# Autodesk Inventor assembly: main_sim
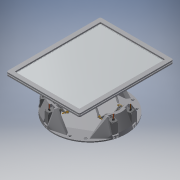
[picture p0: Inventor's stored thumbnail of the model, 180x180]
Saved by Autodesk Inventor 2017 (Build 210142000, 142)
## iProperties
Part Number: main_sim
Material: Ogólny
Document SubType Name: Assembly
Designer: Peter
Author: Peter
## Documents named in this file (5)
- F:\Workspace\Inventor\Ti\CAD\model\Sim assembly\main_sim.iam
- F:\Workspace\Inventor\Ti\CAD\model\Sim assembly\section_lever_sim.ipt
- F:\Workspace\Inventor\Ti\CAD\model\Sim assembly\section_middle_sim.ipt
- F:\Workspace\Inventor\Ti\CAD\model\Sim assembly\section_rod_sim.ipt
- F:\Workspace\Inventor\Ti\CAD\model\Sim assembly\section_upper_sim.ipt
## Components (14 placed, 4 different names)
1. section_middle_sim:1 — Równoległy:2, Równoległy:3, Równoległy:1, Zestawiający:7, Zestawiający:8, Zestawiający:11, Zestawiający:12, Zestawiający:14, Zestawiający:15, Zestawiający:16, Zestawiający:17, Zestawiający:18, Zestawiający:19, Zestawiający:20, Zestawiający:21, Kąt:1, Kąt:2, Kąt:3, Kąt:4, Kąt:5, Kąt:6
2. section_lever_sim:1 — Zestawiający:20, Zestawiający:21, Kąt:1, Zestawiający:22
3. section_lever_sim:2 — Zestawiający:7, Zestawiający:8, Kąt:2, Zestawiający:23
4. section_lever_sim:3 — Zestawiający:11, Zestawiający:12, Kąt:3, Zestawiający:24
5. section_lever_sim:4 — Zestawiający:14, Zestawiający:15, Kąt:4, Zestawiający:25
6. section_lever_sim:5 — Zestawiający:16, Zestawiający:17, Kąt:5, Zestawiający:26
7. section_lever_sim:6 — Zestawiający:18, Zestawiający:19, Kąt:6, Zestawiający:27
8. section_rod_sim:1 — Zestawiający:22, Zestawiający:28
9. section_rod_sim:2 — Zestawiający:23, Zestawiający:29
10. section_rod_sim:3 — Zestawiający:24, Zestawiający:30
11. section_rod_sim:4 — Zestawiający:25, Zestawiający:31
12. section_rod_sim:5 — Zestawiający:26, Zestawiający:32
13. section_rod_sim:6 — Zestawiający:27, Zestawiający:33
14. section_upper_sim:1 — Zestawiający:28, Zestawiający:29, Zestawiający:30, Zestawiający:31, Zestawiający:32, Zestawiający:33
## Relationships (33: Mate 24, Angle 6, Flush 3)
- Równoległy:2 [Flush]: section_middle_sim:1
- Równoległy:3 [Flush]: section_middle_sim:1
- Równoległy:1 [Flush]: section_middle_sim:1
- Zestawiający:7 [Mate]: section_middle_sim:1 ↔ section_lever_sim:2
- Zestawiający:8 [Mate]: section_middle_sim:1 ↔ section_lever_sim:2
- Zestawiający:11 [Mate]: section_middle_sim:1 ↔ section_lever_sim:3
- Zestawiający:12 [Mate]: section_middle_sim:1 ↔ section_lever_sim:3
- Zestawiający:14 [Mate]: section_middle_sim:1 ↔ section_lever_sim:4
- Zestawiający:15 [Mate]: section_middle_sim:1 ↔ section_lever_sim:4
- Zestawiający:16 [Mate]: section_middle_sim:1 ↔ section_lever_sim:5
- Zestawiający:17 [Mate]: section_middle_sim:1 ↔ section_lever_sim:5
- Zestawiający:18 [Mate]: section_middle_sim:1 ↔ section_lever_sim:6
- Zestawiający:19 [Mate]: section_middle_sim:1 ↔ section_lever_sim:6
- Zestawiający:20 [Mate]: section_middle_sim:1 ↔ section_lever_sim:1
- Zestawiający:21 [Mate]: section_middle_sim:1 ↔ section_lever_sim:1
- Kąt:1 [Angle] (0 deg): section_middle_sim:1 ↔ section_lever_sim:1
- Kąt:2 [Angle] (180 deg): section_middle_sim:1 ↔ section_lever_sim:2
- Kąt:3 [Angle] (0 deg): section_middle_sim:1 ↔ section_lever_sim:3
- Kąt:4 [Angle] (180 deg): section_middle_sim:1 ↔ section_lever_sim:4
- Kąt:5 [Angle] (0 deg): section_middle_sim:1 ↔ section_lever_sim:5
- Kąt:6 [Angle] (180 deg): section_middle_sim:1 ↔ section_lever_sim:6
- Zestawiający:22 [Mate]: section_lever_sim:1 ↔ section_rod_sim:1
- Zestawiający:23 [Mate]: section_lever_sim:2 ↔ section_rod_sim:2
- Zestawiający:24 [Mate]: section_lever_sim:3 ↔ section_rod_sim:3
- Zestawiający:25 [Mate]: section_lever_sim:4 ↔ section_rod_sim:4
- Zestawiający:26 [Mate]: section_lever_sim:5 ↔ section_rod_sim:5
- Zestawiający:27 [Mate]: section_lever_sim:6 ↔ section_rod_sim:6
- Zestawiający:28 [Mate]: section_rod_sim:1 ↔ section_upper_sim:1
- Zestawiający:29 [Mate]: section_rod_sim:2 ↔ section_upper_sim:1
- Zestawiający:30 [Mate]: section_rod_sim:3 ↔ section_upper_sim:1
- Zestawiający:31 [Mate]: section_rod_sim:4 ↔ section_upper_sim:1
- Zestawiający:32 [Mate]: section_rod_sim:5 ↔ section_upper_sim:1
- Zestawiający:33 [Mate]: section_rod_sim:6 ↔ section_upper_sim:1
